# Autodesk Inventor assembly: Ensamble base + comp
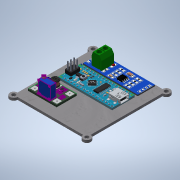
[picture p0: Inventor's stored thumbnail of the model, 180x180]
Saved by Autodesk Inventor 2021 (Build 250183000, 183)
## iProperties
Created: 2021-03-04
Part Number: Ensamble base + comp
Material: Generic
Document SubType Name: Assembly
Designer: Usuario
Author: Usuario
## Documents named in this file (5)
- C:\Users\Usuario\Desktop\INVENTOR\Ensamble base + comp.iam
- C:\Users\Usuario\Desktop\INVENTOR\base.ipt
- C:\Users\Usuario\Desktop\INVENTOR\Arduino\Arduino Nano R3 ATmega 328P.iam
- C:\Users\Usuario\Desktop\INVENTOR\SX1308_STEPUP_DCDC.ipt
- C:\Users\Usuario\Desktop\INVENTOR\rs485.ipt
## Components (4 placed, 4 different names)
1. base:1 — Insert:1, Flush:1, Mate:1, Flush:2, Flush:3, Mate:2
2. Arduino Nano R3 ATmega 328P:1 [sub-assembly] — Insert:1
3. SX1308_STEPUP_DCDC:1 — Flush:3, Mate:2
4. rs485:1 — Flush:1, Mate:1, Flush:2
## Relationships (6: Flush 3, Mate 2, Insert 1)
- Insert:1: base:1 ↔ Arduino Nano R3 ATmega 328P:1
- Flush:1 (1 mm): base:1 ↔ rs485:1
- Mate:1: base:1 ↔ rs485:1
- Flush:2 (8 mm): base:1 ↔ rs485:1
- Flush:3 (3 mm): base:1 ↔ SX1308_STEPUP_DCDC:1
- Mate:2: base:1 ↔ SX1308_STEPUP_DCDC:1
